# Autodesk Inventor assembly: HPTBDW5-SEP
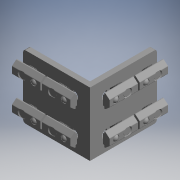
[picture p0: Inventor's stored thumbnail of the model, 180x180]
Saved by Autodesk Inventor 2017.3 (Build 213256000, 256)
## iProperties
Category: PARTsolutions
Company: MISUMI
Part Number: HPTBDW5-SEP
Catalog Web Link: www.cadenas.de
Description: HPTBS5, SHPTBS5, HPTBD5, SHPTBD5, HPTBDW5, SHPTBDW5, HPTGS5-Sheet Metal Brackets - For HFS5 Series - Bent Type
Vendor: MISUMI
Document SubType Name: Assembly
Designer: partserver
Manufacturer: MISUMI
Mass: 14.1348 g
Surface Area: 131.58 cm^2
Volume: 14.1348 cm^3
Density: 1 g/cm^3
Title: HPTBDW5-SEP
Author: Cadenas PARTsolutions
Comments: Sheet Metal Brackets - For HFS5 Series - Bent Type
PSOL_IDENT_0: {$CADENAS_DATA\23d-libs\misumi\metric\38_al_extrusions_blackets\5\hptbs5_asmtab.prj},247 {VTYP=3D},{
PSOL_IDENT_1: STYP=ASSTAB},{NB=HPTBDW5-SEP},{LINA=HPTBDW5-SEP},{NN=HPTBS5, SHPTBS5, HPTBD5, SHPTBD5, HPTBDW5, SHPT
PSOL_IDENT_2: BDW5, HPTGS5},{DATE=08.06.2021 08:25:19},{GEOMDATE=03.04.2020 02:15:02},{VERSION=},{LINEID=270},{WBV
PSOL_IDENT_3: AR=MAT,SHPT,NOH,ALT1},{WBNUMERIC=}  {NB=HPTBDW5-SEP},{LINA=HPTBDW5-SEP},{KT=5},{PN=HPTBDW5-SEP},{TYP
PSOL_IDENT_4: E=HPTBDW},{NO=5},{MAT=},{ST=Trivalent Chromate},{SHPT=L},{SHPTALG= 'L', 'L-Shaped Bent','B', 'Both E
PSOL_IDENT_5: nds Bemt' },{NOH=BDW},{NOHALG= 'BS','2','BD','4','BDW','8' },{MASS=58},{T=3.2},{ALT1=-SEP},{AB=CBM5-
PSOL_IDENT_6: 8},{NOB=8},{AN=HNTP5-5},{NON=8},{AB1=5-8},{AN1=5-5},{MAT1='', 'Low Carbon Steel', 'S', '304 Stainles
PSOL_IDENT_7: s Steel'},{PPATH=hptbs5/hptbs5_asmtpl.prj}
NB: HPTBDW5-SEP
NN: HPTBS5, SHPTBS5, HPTBD5, SHPTBD5, HPTBDW5, SHPTBDW5, HPTGS5
NT: Sheet Metal Brackets - For HFS5 Series - Bent Type
NBSYN: $PN.
LINA: HPTBDW5-SEP
CATALOG: Misumi
PN: HPTBDW5-SEP
NO: 5
MAT: Low Carbon Steel
ST: Trivalent Chromate
SHPT: L-Shaped Bent
NOH: 8
MASS: 58
T: 3.2
ALT1: with SEP (Post-Assembly Fitting Spring Nuts Set of Applicable Bolt and Nut)
AB: CBM5-8
NOB: 8
AN: HNTP5-5
NON: 8
SUPPLIER: MISUMI
ARTICLENO: HPTBDW5-SEP
BOMINFO: HPTBDW5-SEP
CREATOR: CADENAS GmbH
## Documents named in this file (4)
- e:\temp\worker_1\temp\exporttempdir_4700_292_8COVI\format_0\HPTBDW5-SEP.iam
- e:\temp\worker_1\temp\exporttempdir_4700_292_8COVI\format_0\HPTBDW5-SEP_b_.ipt
- e:\temp\worker_1\temp\exporttempdir_4700_292_8COVI\format_0\CBM5-8.ipt
- e:\temp\worker_1\temp\exporttempdir_4700_292_8COVI\format_0\HNTP5-5.ipt
## Components (17 placed, 3 different names)
1. HPTBDW5-SEP_b_:1 — to_cbm_1_1_XY@1 <-> bolt_XY@2, to_cbm_1_1_Z@1 <-> bolt_Z@2, to_cbm_1_1_YZ@1 <-> bolt_YZ@2, to_cbm_1_2_XY@1 <-> bolt_XY@3, to_cbm_1_2_Z@1 <-> bolt_Z@3, to_cbm_1_2_YZ@1 <-> bolt_YZ@3, to_cbm_1_3_XY@1 <-> bolt_XY@4, to_cbm_1_3_Z@1 <-> bolt_Z@4, to_cbm_1_3_YZ@1 <-> bolt_YZ@4, to_cbm_1_4_XY@1 <-> bolt_XY@5, to_cbm_1_4_Z@1 <-> bolt_Z@5, to_cbm_1_4_YZ@1 <-> bolt_YZ@5, to_cbm_2_1_XY@1 <-> bolt_XY@6, to_cbm_2_1_Z@1 <-> bolt_Z@6, to_cbm_2_1_YZ@1 <-> bolt_YZ@6, to_cbm_2_2_XY@1 <-> bolt_XY@7, to_cbm_2_2_Z@1 <-> bolt_Z@7, to_cbm_2_2_YZ@1 <-> bolt_YZ@7, to_cbm_2_3_XY@1 <-> bolt_XY@8, to_cbm_2_3_Z@1 <-> bolt_Z@8, to_cbm_2_3_YZ@1 <-> bolt_YZ@8, to_cbm_2_4_XY@1 <-> bolt_XY@9, to_cbm_2_4_Z@1 <-> bolt_Z@9, to_cbm_2_4_YZ@1 <-> bolt_YZ@9, to_hntp5_1_1_XY@1 <-> to_frames_XY@10, to_hntp5_1_1_Z@1 <-> to_frames_Z@10, to_hntp5_1_1_YZ@1 <-> to_frames_YZ@10, to_hntp5_1_2_XY@1 <-> to_frames_XY@11, to_hntp5_1_2_Z@1 <-> to_frames_Z@11, to_hntp5_1_2_YZ@1 <-> to_frames_YZ@11, to_hntp5_1_3_XY@1 <-> to_frames_XY@12, to_hntp5_1_3_Z@1 <-> to_frames_Z@12, to_hntp5_1_3_YZ@1 <-> to_frames_YZ@12, to_hntp5_1_4_XY@1 <-> to_frames_XY@13, to_hntp5_1_4_Z@1 <-> to_frames_Z@13, to_hntp5_1_4_YZ@1 <-> to_frames_YZ@13, to_hntp5_2_1_XY@1 <-> to_frames_XY@14, to_hntp5_2_1_Z@1 <-> to_frames_Z@14, to_hntp5_2_1_YZ@1 <-> to_frames_YZ@14, to_hntp5_2_2_XY@1 <-> to_frames_XY@15, to_hntp5_2_2_Z@1 <-> to_frames_Z@15, to_hntp5_2_2_YZ@1 <-> to_frames_YZ@15, to_hntp5_2_3_XY@1 <-> to_frames_XY@16, to_hntp5_2_3_Z@1 <-> to_frames_Z@16, to_hntp5_2_3_YZ@1 <-> to_frames_YZ@16, to_hntp5_2_4_XY@1 <-> to_frames_XY@17, to_hntp5_2_4_Z@1 <-> to_frames_Z@17, to_hntp5_2_4_YZ@1 <-> to_frames_YZ@17
2. CBM5-8:1 — to_cbm_1_1_XY@1 <-> bolt_XY@2, to_cbm_1_1_Z@1 <-> bolt_Z@2, to_cbm_1_1_YZ@1 <-> bolt_YZ@2
3. CBM5-8:2 — to_cbm_1_2_XY@1 <-> bolt_XY@3, to_cbm_1_2_Z@1 <-> bolt_Z@3, to_cbm_1_2_YZ@1 <-> bolt_YZ@3
4. CBM5-8:3 — to_cbm_1_3_XY@1 <-> bolt_XY@4, to_cbm_1_3_Z@1 <-> bolt_Z@4, to_cbm_1_3_YZ@1 <-> bolt_YZ@4
5. CBM5-8:4 — to_cbm_1_4_XY@1 <-> bolt_XY@5, to_cbm_1_4_Z@1 <-> bolt_Z@5, to_cbm_1_4_YZ@1 <-> bolt_YZ@5
6. CBM5-8:5 — to_cbm_2_1_XY@1 <-> bolt_XY@6, to_cbm_2_1_Z@1 <-> bolt_Z@6, to_cbm_2_1_YZ@1 <-> bolt_YZ@6
7. CBM5-8:6 — to_cbm_2_2_XY@1 <-> bolt_XY@7, to_cbm_2_2_Z@1 <-> bolt_Z@7, to_cbm_2_2_YZ@1 <-> bolt_YZ@7
8. CBM5-8:7 — to_cbm_2_3_XY@1 <-> bolt_XY@8, to_cbm_2_3_Z@1 <-> bolt_Z@8, to_cbm_2_3_YZ@1 <-> bolt_YZ@8
9. CBM5-8:8 — to_cbm_2_4_XY@1 <-> bolt_XY@9, to_cbm_2_4_Z@1 <-> bolt_Z@9, to_cbm_2_4_YZ@1 <-> bolt_YZ@9
10. HNTP5-5:1 — to_hntp5_1_1_XY@1 <-> to_frames_XY@10, to_hntp5_1_1_Z@1 <-> to_frames_Z@10, to_hntp5_1_1_YZ@1 <-> to_frames_YZ@10
11. HNTP5-5:2 — to_hntp5_1_2_XY@1 <-> to_frames_XY@11, to_hntp5_1_2_Z@1 <-> to_frames_Z@11, to_hntp5_1_2_YZ@1 <-> to_frames_YZ@11
12. HNTP5-5:3 — to_hntp5_1_3_XY@1 <-> to_frames_XY@12, to_hntp5_1_3_Z@1 <-> to_frames_Z@12, to_hntp5_1_3_YZ@1 <-> to_frames_YZ@12
13. HNTP5-5:4 — to_hntp5_1_4_XY@1 <-> to_frames_XY@13, to_hntp5_1_4_Z@1 <-> to_frames_Z@13, to_hntp5_1_4_YZ@1 <-> to_frames_YZ@13
14. HNTP5-5:5 — to_hntp5_2_1_XY@1 <-> to_frames_XY@14, to_hntp5_2_1_Z@1 <-> to_frames_Z@14, to_hntp5_2_1_YZ@1 <-> to_frames_YZ@14
15. HNTP5-5:6 — to_hntp5_2_2_XY@1 <-> to_frames_XY@15, to_hntp5_2_2_Z@1 <-> to_frames_Z@15, to_hntp5_2_2_YZ@1 <-> to_frames_YZ@15
16. HNTP5-5:7 — to_hntp5_2_3_XY@1 <-> to_frames_XY@16, to_hntp5_2_3_Z@1 <-> to_frames_Z@16, to_hntp5_2_3_YZ@1 <-> to_frames_YZ@16
17. HNTP5-5:8 — to_hntp5_2_4_XY@1 <-> to_frames_XY@17, to_hntp5_2_4_Z@1 <-> to_frames_Z@17, to_hntp5_2_4_YZ@1 <-> to_frames_YZ@17
## Relationships (48: Mate 32, Angle 16)
- to_cbm_1_1_XY@1 <-> bolt_XY@2 [Mate]: HPTBDW5-SEP_b_:1 ↔ CBM5-8:1
- to_cbm_1_1_Z@1 <-> bolt_Z@2 [Mate]: HPTBDW5-SEP_b_:1 ↔ CBM5-8:1
- to_cbm_1_1_YZ@1 <-> bolt_YZ@2 [Angle] (0 deg): HPTBDW5-SEP_b_:1 ↔ CBM5-8:1
- to_cbm_1_2_XY@1 <-> bolt_XY@3 [Mate]: HPTBDW5-SEP_b_:1 ↔ CBM5-8:2
- to_cbm_1_2_Z@1 <-> bolt_Z@3 [Mate]: HPTBDW5-SEP_b_:1 ↔ CBM5-8:2
- to_cbm_1_2_YZ@1 <-> bolt_YZ@3 [Angle] (0 deg): HPTBDW5-SEP_b_:1 ↔ CBM5-8:2
- to_cbm_1_3_XY@1 <-> bolt_XY@4 [Mate]: HPTBDW5-SEP_b_:1 ↔ CBM5-8:3
- to_cbm_1_3_Z@1 <-> bolt_Z@4 [Mate]: HPTBDW5-SEP_b_:1 ↔ CBM5-8:3
- to_cbm_1_3_YZ@1 <-> bolt_YZ@4 [Angle] (0 deg): HPTBDW5-SEP_b_:1 ↔ CBM5-8:3
- to_cbm_1_4_XY@1 <-> bolt_XY@5 [Mate]: HPTBDW5-SEP_b_:1 ↔ CBM5-8:4
- to_cbm_1_4_Z@1 <-> bolt_Z@5 [Mate]: HPTBDW5-SEP_b_:1 ↔ CBM5-8:4
- to_cbm_1_4_YZ@1 <-> bolt_YZ@5 [Angle] (0 deg): HPTBDW5-SEP_b_:1 ↔ CBM5-8:4
- to_cbm_2_1_XY@1 <-> bolt_XY@6 [Mate]: HPTBDW5-SEP_b_:1 ↔ CBM5-8:5
- to_cbm_2_1_Z@1 <-> bolt_Z@6 [Mate]: HPTBDW5-SEP_b_:1 ↔ CBM5-8:5
- to_cbm_2_1_YZ@1 <-> bolt_YZ@6 [Angle] (0 deg): HPTBDW5-SEP_b_:1 ↔ CBM5-8:5
- to_cbm_2_2_XY@1 <-> bolt_XY@7 [Mate]: HPTBDW5-SEP_b_:1 ↔ CBM5-8:6
- to_cbm_2_2_Z@1 <-> bolt_Z@7 [Mate]: HPTBDW5-SEP_b_:1 ↔ CBM5-8:6
- to_cbm_2_2_YZ@1 <-> bolt_YZ@7 [Angle] (0 deg): HPTBDW5-SEP_b_:1 ↔ CBM5-8:6
- to_cbm_2_3_XY@1 <-> bolt_XY@8 [Mate]: HPTBDW5-SEP_b_:1 ↔ CBM5-8:7
- to_cbm_2_3_Z@1 <-> bolt_Z@8 [Mate]: HPTBDW5-SEP_b_:1 ↔ CBM5-8:7
- to_cbm_2_3_YZ@1 <-> bolt_YZ@8 [Angle] (0 deg): HPTBDW5-SEP_b_:1 ↔ CBM5-8:7
- to_cbm_2_4_XY@1 <-> bolt_XY@9 [Mate]: HPTBDW5-SEP_b_:1 ↔ CBM5-8:8
- to_cbm_2_4_Z@1 <-> bolt_Z@9 [Mate]: HPTBDW5-SEP_b_:1 ↔ CBM5-8:8
- to_cbm_2_4_YZ@1 <-> bolt_YZ@9 [Angle] (0 deg): HPTBDW5-SEP_b_:1 ↔ CBM5-8:8
- to_hntp5_1_1_XY@1 <-> to_frames_XY@10 [Mate]: HPTBDW5-SEP_b_:1 ↔ HNTP5-5:1
- to_hntp5_1_1_Z@1 <-> to_frames_Z@10 [Mate]: HPTBDW5-SEP_b_:1 ↔ HNTP5-5:1
- to_hntp5_1_1_YZ@1 <-> to_frames_YZ@10 [Angle] (0 deg): HPTBDW5-SEP_b_:1 ↔ HNTP5-5:1
- to_hntp5_1_2_XY@1 <-> to_frames_XY@11 [Mate]: HPTBDW5-SEP_b_:1 ↔ HNTP5-5:2
- to_hntp5_1_2_Z@1 <-> to_frames_Z@11 [Mate]: HPTBDW5-SEP_b_:1 ↔ HNTP5-5:2
- to_hntp5_1_2_YZ@1 <-> to_frames_YZ@11 [Angle] (0 deg): HPTBDW5-SEP_b_:1 ↔ HNTP5-5:2
- to_hntp5_1_3_XY@1 <-> to_frames_XY@12 [Mate]: HPTBDW5-SEP_b_:1 ↔ HNTP5-5:3
- to_hntp5_1_3_Z@1 <-> to_frames_Z@12 [Mate]: HPTBDW5-SEP_b_:1 ↔ HNTP5-5:3
- to_hntp5_1_3_YZ@1 <-> to_frames_YZ@12 [Angle] (0 deg): HPTBDW5-SEP_b_:1 ↔ HNTP5-5:3
- to_hntp5_1_4_XY@1 <-> to_frames_XY@13 [Mate]: HPTBDW5-SEP_b_:1 ↔ HNTP5-5:4
- to_hntp5_1_4_Z@1 <-> to_frames_Z@13 [Mate]: HPTBDW5-SEP_b_:1 ↔ HNTP5-5:4
- to_hntp5_1_4_YZ@1 <-> to_frames_YZ@13 [Angle] (0 deg): HPTBDW5-SEP_b_:1 ↔ HNTP5-5:4
- to_hntp5_2_1_XY@1 <-> to_frames_XY@14 [Mate]: HPTBDW5-SEP_b_:1 ↔ HNTP5-5:5
- to_hntp5_2_1_Z@1 <-> to_frames_Z@14 [Mate]: HPTBDW5-SEP_b_:1 ↔ HNTP5-5:5
- to_hntp5_2_1_YZ@1 <-> to_frames_YZ@14 [Angle] (0 deg): HPTBDW5-SEP_b_:1 ↔ HNTP5-5:5
- to_hntp5_2_2_XY@1 <-> to_frames_XY@15 [Mate]: HPTBDW5-SEP_b_:1 ↔ HNTP5-5:6
- to_hntp5_2_2_Z@1 <-> to_frames_Z@15 [Mate]: HPTBDW5-SEP_b_:1 ↔ HNTP5-5:6
- to_hntp5_2_2_YZ@1 <-> to_frames_YZ@15 [Angle] (0 deg): HPTBDW5-SEP_b_:1 ↔ HNTP5-5:6
- to_hntp5_2_3_XY@1 <-> to_frames_XY@16 [Mate]: HPTBDW5-SEP_b_:1 ↔ HNTP5-5:7
- to_hntp5_2_3_Z@1 <-> to_frames_Z@16 [Mate]: HPTBDW5-SEP_b_:1 ↔ HNTP5-5:7
- to_hntp5_2_3_YZ@1 <-> to_frames_YZ@16 [Angle] (0 deg): HPTBDW5-SEP_b_:1 ↔ HNTP5-5:7
- to_hntp5_2_4_XY@1 <-> to_frames_XY@17 [Mate]: HPTBDW5-SEP_b_:1 ↔ HNTP5-5:8
- to_hntp5_2_4_Z@1 <-> to_frames_Z@17 [Mate]: HPTBDW5-SEP_b_:1 ↔ HNTP5-5:8
- to_hntp5_2_4_YZ@1 <-> to_frames_YZ@17 [Angle] (0 deg): HPTBDW5-SEP_b_:1 ↔ HNTP5-5:8
